# Autodesk Inventor assembly: A102EnsembleCamera
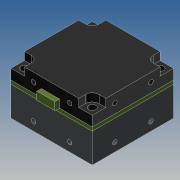
[picture p0: Inventor's stored thumbnail of the model, 180x180]
Saved by Autodesk Inventor 2017 (Build 210142000, 142)
## iProperties
Created: 2016-10-19
Part Number: A102EnsembleCamera
Document SubType Name: Assembly
Designer: serge.amoos
Author: serge.amoos
## Documents named in this file (4)
- I:\RaD\SI-ET\Projets\51346-SmartLens\inventor\FocalMeasure\A102EnsembleCamera.iam
- I:\RaD\SI-ET\Projets\51346-SmartLens\inventor\FocalMeasure\P106BoitierCameraArriere.ipt
- I:\RaD\SI-ET\Projets\51346-SmartLens\inventor\FocalMeasure\F103CameraUsb.ipt
- I:\RaD\SI-ET\Projets\51346-SmartLens\inventor\FocalMeasure\P107BoitierCameraAvant.ipt
## Components (3 placed, 3 different names)
1. P106BoitierCameraArriere:1 — Mate:1, Mate:2, Mate:3, Mate:5, Mate:6
2. F103CameraUsb:1 — Mate:1, Mate:2, Mate:3, Mate:4
3. P107BoitierCameraAvant:1 — Mate:4, Mate:5, Mate:6
## Relationships (6: Mate 6)
- Mate:1: P106BoitierCameraArriere:1 ↔ F103CameraUsb:1
- Mate:2: P106BoitierCameraArriere:1 ↔ F103CameraUsb:1
- Mate:3: P106BoitierCameraArriere:1 ↔ F103CameraUsb:1
- Mate:4: F103CameraUsb:1 ↔ P107BoitierCameraAvant:1
- Mate:5: P106BoitierCameraArriere:1 ↔ P107BoitierCameraAvant:1
- Mate:6: P106BoitierCameraArriere:1 ↔ P107BoitierCameraAvant:1
